# Autodesk Inventor assembly: Robot_Arm
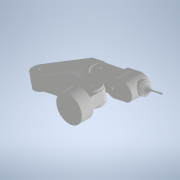
[picture p0: Inventor's stored thumbnail of the model, 180x180]
Saved by Autodesk Inventor 2021 (Build 250183000, 183)
## iProperties
Created: 2024-09-30
Part Number: Robot_Arm
Document SubType Name: Assembly
Designer: Swoby
Author: Swoby
## Documents named in this file (8)
- C:\Users\Swoby\OneDrive\Plocha\DUM-E\V0.3\Overeni_Matlab\Inventor 2021 zjednoduseny model\Robot_Arm.iam
- C:\Users\Swoby\OneDrive\Plocha\DUM-E\V0.3\Overeni_Matlab\Inventor 2021 zjednoduseny model\Base.ipt
- C:\Users\Swoby\OneDrive\Plocha\DUM-E\V0.3\Overeni_Matlab\Inventor 2021 zjednoduseny model\Base2.ipt
- C:\Users\Swoby\OneDrive\Plocha\DUM-E\V0.3\Overeni_Matlab\Inventor 2021 zjednoduseny model\Arm1.ipt
- C:\Users\Swoby\OneDrive\Plocha\DUM-E\V0.3\Overeni_Matlab\Inventor 2021 zjednoduseny model\Arm2.ipt
- C:\Users\Swoby\OneDrive\Plocha\DUM-E\V0.3\Overeni_Matlab\Inventor 2021 zjednoduseny model\Wirst1.ipt
- C:\Users\Swoby\OneDrive\Plocha\DUM-E\V0.3\Overeni_Matlab\Inventor 2021 zjednoduseny model\Wirst2.ipt
- C:\Users\Swoby\OneDrive\Plocha\DUM-E\V0.3\Overeni_Matlab\Inventor 2021 zjednoduseny model\EndEffector.ipt
## Components (7 placed, 7 different names)
1. Base:1 — Mate:1, Mate:2
2. Base2:1 — Mate:1, Mate:2, Mate:3, Mate:4
3. Arm1:1 — Mate:3, Mate:4, Mate:5, Mate:6
4. Arm2:1 — Mate:5, Mate:6, Mate:7, Mate:8
5. Wirst1:1 — Mate:7, Mate:8, Mate:9, Mate:10
6. Wirst2:1 — Mate:9, Mate:10, Mate:11, Mate:12
7. EndEffector:1 — Mate:11, Mate:12
## Relationships (12: Mate 12)
- Mate:1: Base:1 ↔ Base2:1
- Mate:2: Base:1 ↔ Base2:1
- Mate:3: Base2:1 ↔ Arm1:1
- Mate:4: Base2:1 ↔ Arm1:1
- Mate:5: Arm1:1 ↔ Arm2:1
- Mate:6: Arm1:1 ↔ Arm2:1
- Mate:7: Arm2:1 ↔ Wirst1:1
- Mate:8: Arm2:1 ↔ Wirst1:1
- Mate:9: Wirst1:1 ↔ Wirst2:1
- Mate:10: Wirst1:1 ↔ Wirst2:1
- Mate:11: Wirst2:1 ↔ EndEffector:1
- Mate:12: Wirst2:1 ↔ EndEffector:1
